# Autodesk Inventor assembly: pulley-belt
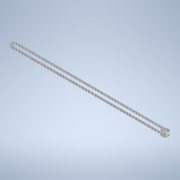
[picture p0: Inventor's stored thumbnail of the model, 180x180]
Saved by Autodesk Inventor 2020 (Build 240168000, 168)
## iProperties
Created: 2021-02-20
Part Number: pulley-belt
Document SubType Name: Assembly
Designer: AOB
Mass: 5.91044 g
Surface Area: 139.989 cm^2
Volume: 4.11036 cm^3
Density: 1.43794 g/cm^3
Author: AOB
## Documents named in this file (4)
- C:\Users\marti\Documents\Inventor\ProjectBoron\pulley-belt.iam
- C:\Users\marti\Documents\Inventor\ProjectBoron\pulley.ipt
- C:\Users\marti\Documents\Inventor\ProjectBoron\belt-outline.ipt
- C:\Users\marti\Documents\Inventor\ProjectBoron\gt2-2.ipt
## Components (428 placed, 3 different names)
1. pulley:2 — Mate:3
2. belt-outline:1 — Flush:1, Flush:2, Flush:3, Flush:4, Mate:1, Mate:3
3. gt2-2:1 — Flush:4, Mate:1, Angle:1, Angle:2, Angle:3
4. gt2-2:2
5. gt2-2:3
6. gt2-2:4
7. gt2-2:5
8. gt2-2:6
9. gt2-2:7
10. gt2-2:8 — Symmetry:1
11. gt2-2:9 — Symmetry:1
12. gt2-2:10
13. gt2-2:11
14. gt2-2:12
15. gt2-2:13
16. gt2-2:14
17. gt2-2:15
18. gt2-2:16
19. gt2-2:17
20. gt2-2:18
21. gt2-2:19
22. gt2-2:20
23. gt2-2:21
24. gt2-2:22
25. gt2-2:23
26. gt2-2:24
27. gt2-2:25
28. gt2-2:26
29. gt2-2:27
30. gt2-2:28
31. gt2-2:29
32. gt2-2:30
33. gt2-2:31
34. gt2-2:32
35. gt2-2:33
36. gt2-2:34
37. gt2-2:35
38. gt2-2:36
39. gt2-2:37
40. gt2-2:38
41. gt2-2:39
42. gt2-2:40
43. gt2-2:41
44. gt2-2:42
45. gt2-2:43
46. gt2-2:44
47. gt2-2:45
48. gt2-2:46
49. gt2-2:47
50. gt2-2:48
51. gt2-2:49
52. gt2-2:50
53. gt2-2:51
54. gt2-2:52
55. gt2-2:53
56. gt2-2:54
57. gt2-2:55
58. gt2-2:56
59. gt2-2:57
60. gt2-2:58
61. gt2-2:59
62. gt2-2:60
63. gt2-2:61
64. gt2-2:62
65. gt2-2:63
66. gt2-2:64
67. gt2-2:65
68. gt2-2:66
69. gt2-2:67
70. gt2-2:68
71. gt2-2:69
72. gt2-2:70
73. gt2-2:71
74. gt2-2:72
75. gt2-2:73
76. gt2-2:74
77. gt2-2:75
78. gt2-2:76
79. gt2-2:77
80. gt2-2:78
81. gt2-2:79
82. gt2-2:80
83. gt2-2:81
84. gt2-2:82
85. gt2-2:83
86. gt2-2:84
87. gt2-2:85
88. gt2-2:86
89. gt2-2:87
90. gt2-2:88
91. gt2-2:89
92. gt2-2:90
93. gt2-2:91
94. gt2-2:92
95. gt2-2:93
96. gt2-2:94
97. gt2-2:95
98. gt2-2:96
99. gt2-2:97
100. gt2-2:98
101. gt2-2:99
102. gt2-2:100
103. gt2-2:101
104. gt2-2:102
105. gt2-2:103
106. gt2-2:104
107. gt2-2:105
108. gt2-2:106
109. gt2-2:107
110. gt2-2:108
111. gt2-2:109
112. gt2-2:110
113. gt2-2:111
114. gt2-2:112
115. gt2-2:113
116. gt2-2:114
117. gt2-2:115
118. gt2-2:116
119. gt2-2:117
120. gt2-2:118
121. gt2-2:119
122. gt2-2:120
123. gt2-2:121
124. gt2-2:122
125. gt2-2:123
126. gt2-2:124
127. gt2-2:125
128. gt2-2:126
129. gt2-2:127
130. gt2-2:128
131. gt2-2:129
132. gt2-2:130
133. gt2-2:131
134. gt2-2:132
135. gt2-2:133
136. gt2-2:134
137. gt2-2:135
138. gt2-2:136
139. gt2-2:137
140. gt2-2:138
141. gt2-2:139
142. gt2-2:140
143. gt2-2:141
144. gt2-2:142
145. gt2-2:143
146. gt2-2:144
147. gt2-2:145
148. gt2-2:146
149. gt2-2:147
150. gt2-2:148
151. gt2-2:149
152. gt2-2:150
153. gt2-2:151
154. gt2-2:152
155. gt2-2:153
156. gt2-2:154
157. gt2-2:155
158. gt2-2:156
159. gt2-2:157
160. gt2-2:158
161. gt2-2:159
162. gt2-2:160
163. gt2-2:161
164. gt2-2:162
165. gt2-2:163
166. gt2-2:164
167. gt2-2:165
168. gt2-2:166
169. gt2-2:167
170. gt2-2:168
171. gt2-2:169
172. gt2-2:170
173. gt2-2:171
174. gt2-2:172
175. gt2-2:173
176. gt2-2:174
177. gt2-2:175
178. gt2-2:176
179. gt2-2:177
180. gt2-2:178
181. gt2-2:179
182. gt2-2:180
183. gt2-2:181
184. gt2-2:182
185. gt2-2:183
186. gt2-2:184
187. gt2-2:185
188. gt2-2:186
189. gt2-2:187
190. gt2-2:188
191. gt2-2:189
192. gt2-2:190
193. gt2-2:191
194. gt2-2:192
195. gt2-2:193
196. gt2-2:194
197. gt2-2:195
198. gt2-2:196
199. gt2-2:197
200. gt2-2:198
201. gt2-2:199
202. gt2-2:200
203. gt2-2:201
204. gt2-2:202
205. gt2-2:203
206. gt2-2:204
207. gt2-2:205
208. gt2-2:206
209. gt2-2:207
210. gt2-2:208
211. gt2-2:209
212. gt2-2:210
213. gt2-2:211
214. gt2-2:212
215. gt2-2:213
216. gt2-2:214
217. gt2-2:215
218. gt2-2:216
219. gt2-2:217
220. gt2-2:218
221. gt2-2:219
222. gt2-2:220
223. gt2-2:221
224. gt2-2:222
225. gt2-2:223
226. gt2-2:224
227. gt2-2:225
228. gt2-2:226
229. gt2-2:227
230. gt2-2:228
231. gt2-2:229
232. gt2-2:230
233. gt2-2:231
234. gt2-2:232
235. gt2-2:233
236. gt2-2:234
237. gt2-2:235
238. gt2-2:236
239. gt2-2:237
240. gt2-2:238
241. gt2-2:239
242. gt2-2:240
243. gt2-2:241
244. gt2-2:242
245. gt2-2:243
246. gt2-2:244
247. gt2-2:245
248. gt2-2:246
249. gt2-2:247
250. gt2-2:248
251. gt2-2:249
252. gt2-2:250
253. gt2-2:251
254. gt2-2:252
255. gt2-2:253
256. gt2-2:254
257. gt2-2:255
258. gt2-2:256
259. gt2-2:257
260. gt2-2:258
261. gt2-2:259
262. gt2-2:260
263. gt2-2:261
264. gt2-2:262
265. gt2-2:263
266. gt2-2:264
267. gt2-2:265
268. gt2-2:266
269. gt2-2:267
270. gt2-2:268
271. gt2-2:269
272. gt2-2:270
273. gt2-2:271
274. gt2-2:272
275. gt2-2:273
276. gt2-2:274
277. gt2-2:275
278. gt2-2:276
279. gt2-2:277
280. gt2-2:278
281. gt2-2:279
282. gt2-2:280
283. gt2-2:281
284. gt2-2:282
285. gt2-2:283
286. gt2-2:284
287. gt2-2:285
288. gt2-2:286
289. gt2-2:287
290. gt2-2:288
291. gt2-2:289
292. gt2-2:290
293. gt2-2:291
294. gt2-2:292
295. gt2-2:293
296. gt2-2:294
297. gt2-2:295
298. gt2-2:296
299. gt2-2:297
300. gt2-2:298
301. gt2-2:299
302. gt2-2:300
303. gt2-2:301
304. gt2-2:302
305. gt2-2:303
306. gt2-2:304
307. gt2-2:305
308. gt2-2:306
309. gt2-2:307
310. gt2-2:308
311. gt2-2:309
312. gt2-2:310
313. gt2-2:311
314. gt2-2:312
315. gt2-2:313
316. gt2-2:314
317. gt2-2:315
318. gt2-2:316
319. gt2-2:317
320. gt2-2:318
321. gt2-2:319
322. gt2-2:320
323. gt2-2:321
324. gt2-2:322
325. gt2-2:323
326. gt2-2:324
327. gt2-2:325
328. gt2-2:326
329. gt2-2:327
330. gt2-2:328
331. gt2-2:329
332. gt2-2:330
333. gt2-2:331
334. gt2-2:332
335. gt2-2:333
336. gt2-2:334
337. gt2-2:335
338. gt2-2:336
339. gt2-2:337
340. gt2-2:338
341. gt2-2:339
342. gt2-2:340
343. gt2-2:341
344. gt2-2:342
345. gt2-2:343
346. gt2-2:344
347. gt2-2:345
348. gt2-2:346
349. gt2-2:347
350. gt2-2:348
351. gt2-2:349
352. gt2-2:350
353. gt2-2:351
354. gt2-2:352
355. gt2-2:353
356. gt2-2:354
357. gt2-2:355
358. gt2-2:356
359. gt2-2:357
360. gt2-2:358
361. gt2-2:359
362. gt2-2:360
363. gt2-2:361
364. gt2-2:362
365. gt2-2:363
366. gt2-2:364
367. gt2-2:365
368. gt2-2:366
369. gt2-2:367
370. gt2-2:368
371. gt2-2:369
372. gt2-2:370
373. gt2-2:371
374. gt2-2:372
375. gt2-2:373
376. gt2-2:374
377. gt2-2:375
378. gt2-2:376
379. gt2-2:377
380. gt2-2:378
381. gt2-2:379
382. gt2-2:380
383. gt2-2:381
384. gt2-2:382
385. gt2-2:383
386. gt2-2:384
387. gt2-2:385
388. gt2-2:386
389. gt2-2:387
390. gt2-2:388
391. gt2-2:389
392. gt2-2:390
393. gt2-2:391
394. gt2-2:392
395. gt2-2:393
396. gt2-2:394
397. gt2-2:395
398. gt2-2:396
399. gt2-2:397
400. gt2-2:398
401. gt2-2:399
402. gt2-2:400
403. gt2-2:401
404. gt2-2:402
405. gt2-2:403
406. gt2-2:404
407. gt2-2:405
408. gt2-2:406
409. gt2-2:407
410. gt2-2:408
411. gt2-2:409
412. gt2-2:410
413. gt2-2:411
414. gt2-2:412
415. gt2-2:413
416. gt2-2:414
417. gt2-2:415
418. gt2-2:416
419. gt2-2:417
420. gt2-2:418
421. gt2-2:419
422. gt2-2:420
423. gt2-2:421
424. gt2-2:422
425. gt2-2:423
426. gt2-2:424
427. gt2-2:425
428. gt2-2:426
## Component patterns: (426 elements, first: gt2-2:1)
## Relationships (12: Flush 5, Mate 3, Angle 3, Symmetry 1)
- Flush:1: belt-outline:1
- Flush:2: belt-outline:1
- Flush:3: belt-outline:1
- Flush:4: belt-outline:1 ↔ gt2-2:1
- Mate:1: belt-outline:1 ↔ gt2-2:1
- Angle:1 (0 deg): gt2-2:1
- Angle:2 (0 deg): gt2-2:1
- Angle:3 (0 deg): gt2-2:1
- Symmetry:1: gt2-2:8 ↔ gt2-2:9
- Flush:6
- Mate:3: pulley:2 ↔ belt-outline:1
- Mate:4
